# Autodesk Inventor assembly: am-2598_1072016KOPToughboxMini_1
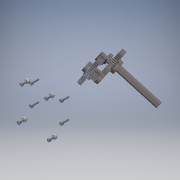
[picture p0: Inventor's stored thumbnail of the model, 180x180]
Saved by Autodesk Inventor 2018 (Build 220112000, 112)
## iProperties
Created: 2017-01-13
Part Number: am-2598_1072016KOPToughboxMini_1
Description: STEP AP214
Document SubType Name: Assembly
Designer: lopez.xavier
Sending System: SolidWorks 2014
Preprocessor: SwSTEP 2.0
Title: am-2598_107 2016 KOP Toughbox Mini.STEP
Revision Number: ANY
## Documents named in this file (16)
- C:\Users\lopez.xavier\Downloads\am-2598_1072016KOPToughboxMini_1.iam
- C:\Users\lopez.xavier\Downloads\Toughbox d07.ipt
- C:\Users\lopez.xavier\Downloads\Toughbox d05.ipt
- C:\Users\lopez.xavier\Downloads\FR6ZZ Bearing.ipt
- C:\Users\lopez.xavier\Downloads\10-32 Nylock Nut.ipt
- C:\Users\lopez.xavier\Downloads\5-16 washer.ipt
- C:\Users\lopez.xavier\Downloads\Toughbox d09.ipt
- C:\Users\lopez.xavier\Downloads\TM Housing.ipt
- C:\Users\lopez.xavier\Downloads\SHCS 10-32 x 0.625.ipt
- C:\Users\lopez.xavier\Downloads\R6ZZ Bearing.ipt
- C:\Users\lopez.xavier\Downloads\8mm spring clip.ipt
- C:\Users\lopez.xavier\Downloads\500 E-klip.ipt
- C:\Users\lopez.xavier\Downloads\FR8ZZ Hex Bearing.ipt
- C:\Users\lopez.xavier\Downloads\16t 20dp 375h with teeth.ipt
- C:\Users\lopez.xavier\Downloads\48t 20dp 500h with teeth.ipt
- C:\Users\lopez.xavier\Downloads\TB Output Shaft Hex L-Base 2.ipt
## Components (31 placed, 31 different names)
1. Toughbox d07_1 — Insert:1, Mate:8, Mate:9, Mate:11, Mate:12, Mate:48
2. Toughbox d05_2 — Mate:8, Mate:9, Mate:10, Mate:13, Mate:32
3. 10-32 Nylock Nut_4
4. 10-32 Nylock Nut_5
5. 10-32 Nylock Nut_6
6. 10-32 Nylock Nut_7
7. 5-16 washer_8 — Mate:55, Mate:56
8. 5-16 washer_9 — Mate:41, Mate:42, Mate:51, Mate:54, Mate:57
9. 5-16 washer_10 — Mate:54, Mate:57
10. 5-16 washer_11 — Mate:40, Mate:43, Mate:53, Mate:55, Mate:56
11. Toughbox d09_12 — Mate:41, Mate:42, Mate:44, Mate:45, Mate:50
12. Toughbox d09_13 — Mate:40, Mate:43, Mate:46, Mate:47, Mate:52
13. TM Housing_14 — Mate:38, Mate:39, Mate:50, Mate:51, Mate:52, Mate:53, Mate:58, Mate:59
14. SHCS 10-32 x 0.625_15
15. SHCS 10-32 x 0.625_16
16. SHCS 10-32 x 0.625_17
17. SHCS 10-32 x 0.625_18
18. SHCS 10-32 x 0.625_19
19. SHCS 10-32 x 0.625_20
20. SHCS 10-32 x 0.625_21
21. SHCS 10-32 x 0.625_22
22. R6ZZ Bearing_23 — Insert:1, Mate:10, Mate:58, Mate:59
23. R6ZZ Bearing_24 — Mate:16, Mate:17
24. 8mm spring clip_25 — Mate:46, Mate:47
25. 8mm spring clip_26 — Mate:44, Mate:45
26. 500 E-klip_27 — Mate:18, Mate:19, Mate:25, Mate:26
27. FR8ZZ Hex Bearing_28 — Mate:26, Mate:28, Mate:29
28. 16t 20dp 375h with teeth_29 — Mate:11, Mate:12, Mate:13, Mate:32, Mate:49
29. 48t 20dp 500h with teeth_30 — Mate:25, Mate:27, Mate:30, Mate:31
30. TB Output Shaft Hex L-Base 2_31 — Mate:16, Mate:17, Mate:18, Mate:19, Mate:27, Mate:28, Mate:29, Mate:30, Mate:31, Mate:38, Mate:39
31. FR6ZZ Bearing:1 — Mate:48, Mate:49
## Relationships (41: Mate 40, Insert 1)
- Insert:1: Toughbox d07_1 ↔ R6ZZ Bearing_23
- Mate:8: Toughbox d07_1 ↔ Toughbox d05_2
- Mate:9: Toughbox d07_1 ↔ Toughbox d05_2
- Mate:10: Toughbox d05_2 ↔ R6ZZ Bearing_23
- Mate:11: Toughbox d07_1 ↔ 16t 20dp 375h with teeth_29
- Mate:12: Toughbox d07_1 ↔ 16t 20dp 375h with teeth_29
- Mate:13: Toughbox d05_2 ↔ 16t 20dp 375h with teeth_29
- Mate:16: R6ZZ Bearing_24 ↔ TB Output Shaft Hex L-Base 2_31
- Mate:17: R6ZZ Bearing_24 ↔ TB Output Shaft Hex L-Base 2_31
- Mate:18: 500 E-klip_27 ↔ TB Output Shaft Hex L-Base 2_31
- Mate:19: 500 E-klip_27 ↔ TB Output Shaft Hex L-Base 2_31
- Mate:25: 500 E-klip_27 ↔ 48t 20dp 500h with teeth_30
- Mate:26: 500 E-klip_27 ↔ FR8ZZ Hex Bearing_28
- Mate:27: 48t 20dp 500h with teeth_30 ↔ TB Output Shaft Hex L-Base 2_31
- Mate:28: FR8ZZ Hex Bearing_28 ↔ TB Output Shaft Hex L-Base 2_31
- Mate:29: FR8ZZ Hex Bearing_28 ↔ TB Output Shaft Hex L-Base 2_31
- Mate:30: 48t 20dp 500h with teeth_30 ↔ TB Output Shaft Hex L-Base 2_31
- Mate:31: 48t 20dp 500h with teeth_30 ↔ TB Output Shaft Hex L-Base 2_31
- Mate:32: Toughbox d05_2 ↔ 16t 20dp 375h with teeth_29
- Mate:38: TM Housing_14 ↔ TB Output Shaft Hex L-Base 2_31
- Mate:39: TM Housing_14 ↔ TB Output Shaft Hex L-Base 2_31
- Mate:40: 5-16 washer_11 ↔ Toughbox d09_13
- Mate:41: 5-16 washer_9 ↔ Toughbox d09_12
- Mate:42: 5-16 washer_9 ↔ Toughbox d09_12
- Mate:43: 5-16 washer_11 ↔ Toughbox d09_13
- Mate:44: Toughbox d09_12 ↔ 8mm spring clip_26
- Mate:45: Toughbox d09_12 ↔ 8mm spring clip_26
- Mate:46: Toughbox d09_13 ↔ 8mm spring clip_25
- Mate:47: Toughbox d09_13 ↔ 8mm spring clip_25
- Mate:48: Toughbox d07_1 ↔ FR6ZZ Bearing:1
- Mate:49: 16t 20dp 375h with teeth_29 ↔ FR6ZZ Bearing:1
- Mate:50: Toughbox d09_12 ↔ TM Housing_14
- Mate:51: 5-16 washer_9 ↔ TM Housing_14
- Mate:52: Toughbox d09_13 ↔ TM Housing_14
- Mate:53: 5-16 washer_11 ↔ TM Housing_14
- Mate:54: 5-16 washer_9 ↔ 5-16 washer_10
- Mate:55: 5-16 washer_8 ↔ 5-16 washer_11
- Mate:56: 5-16 washer_8 ↔ 5-16 washer_11
- Mate:57: 5-16 washer_9 ↔ 5-16 washer_10
- Mate:58: TM Housing_14 ↔ R6ZZ Bearing_23
- Mate:59 (-7.62 mm): TM Housing_14 ↔ R6ZZ Bearing_23
